# Autodesk Inventor assembly: OkiagariKoboshi
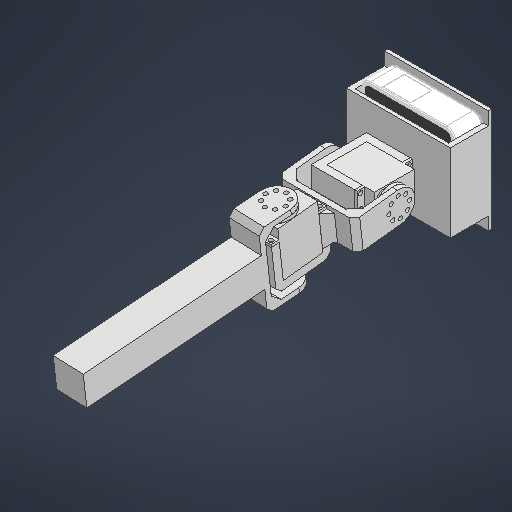
[picture p0: Inventor's stored thumbnail of the model, 512x512]
Saved by Autodesk Inventor 2026 (Build 300175050, 175E)
## iProperties
Created: 2026-07-07
Part Number: OkiagariKoboshi
Document SubType Name: Assembly
Designer: hanaj
Author: hanaj
## Documents named in this file (7)
- C:\Users\hanaj\OkiagariKoboshi_ws\CAD\OkiagariKoboshi.iam
- C:\Users\hanaj\OkiagariKoboshi_ws\CAD\M5Stack_Core2\M5Stack_Core2\M5Stack_Core2.ipt
- C:\Users\hanaj\OkiagariKoboshi_ws\CAD\STS3032.ipt
- C:\Users\hanaj\OkiagariKoboshi_ws\CAD\STS3032_Horn.ipt
- C:\Users\hanaj\OkiagariKoboshi_ws\CAD\Base.ipt
- C:\Users\hanaj\OkiagariKoboshi_ws\CAD\Arm1.ipt
- C:\Users\hanaj\OkiagariKoboshi_ws\CAD\Arm2.ipt
## Components (8 placed, 6 different names)
1. M5Stack_Core2:1 — メイト:3
2. STS3032:1 — メイト:4, メイト:5, フラッシュ:1, 円柱状:1, メイト:9
3. STS3032_Horn:1 — 円柱状:1, メイト:9, メイト:10, メイト:11, メイト:12
4. Base:1 — メイト:3, メイト:4, メイト:5, フラッシュ:1
5. Arm1:1 — メイト:7, メイト:8, フラッシュ:2, メイト:10, メイト:11, メイト:12
6. STS3032:2 — メイト:7, メイト:8, フラッシュ:2, 円柱状:2, メイト:13
7. STS3032_Horn:2 — 円柱状:2, メイト:13, メイト:14, メイト:15, メイト:16
8. Arm2:1 — メイト:14, メイト:15, メイト:16
## Relationships (17: Mate 13, Flush 2, CylindricalJoint 2)
- メイト:3 [Mate]: M5Stack_Core2:1 ↔ Base:1
- メイト:4 [Mate]: STS3032:1 ↔ Base:1
- メイト:5 [Mate]: STS3032:1 ↔ Base:1
- フラッシュ:1 [Flush]: STS3032:1 ↔ Base:1
- メイト:7 [Mate]: Arm1:1 ↔ STS3032:2
- メイト:8 [Mate]: Arm1:1 ↔ STS3032:2
- フラッシュ:2 [Flush]: Arm1:1 ↔ STS3032:2
- 円柱状:1 [CylindricalJoint]: STS3032:1 ↔ STS3032_Horn:1
- メイト:9 [Mate]: STS3032:1 ↔ STS3032_Horn:1
- メイト:10 [Mate]: STS3032_Horn:1 ↔ Arm1:1
- メイト:11 [Mate]: STS3032_Horn:1 ↔ Arm1:1
- メイト:12 [Mate]: STS3032_Horn:1 ↔ Arm1:1
- 円柱状:2 [CylindricalJoint]: STS3032:2 ↔ STS3032_Horn:2
- メイト:13 [Mate]: STS3032:2 ↔ STS3032_Horn:2
- メイト:14 [Mate]: STS3032_Horn:2 ↔ Arm2:1
- メイト:15 [Mate]: STS3032_Horn:2 ↔ Arm2:1
- メイト:16 [Mate]: STS3032_Horn:2 ↔ Arm2:1
